# Autodesk Inventor assembly: !drive_pod
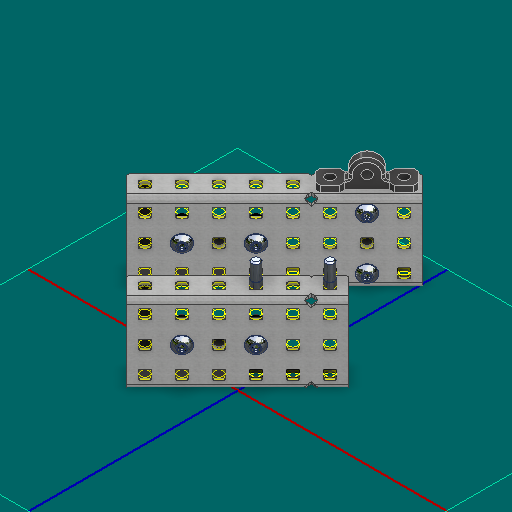
[picture p0: Inventor's stored thumbnail of the model, 512x512]
Saved by Autodesk Inventor 2025 (Build 290162000, 162)
## iProperties
Created: 2024-08-16
Part Number: !drive_pod
Document SubType Name: Assembly
Designer: averey
Author: averey
## Documents named in this file (12)
- C:\Users\avere\vex_robotics_high_stakes\hardware\cad\ATLAS\chassis\drive_pod\structure.iam
- C:\Users\avere\vex_robotics_high_stakes\hardware\cad\VEX-CAD-Inventor\Structure\C Channel\Aluminum 1x3x1\Alu C 1x3x1x6.ipt
- C:\Users\avere\vex_robotics_high_stakes\hardware\cad\_quick_assemblies\bearing_flat_w_hardware.iam
- C:\Users\avere\vex_robotics_high_stakes\hardware\cad\VEX-CAD-Inventor\Structure\C Channel\Aluminum 1x3x1\Alu C 1x3x1x8.ipt
- C:\Users\avere\vex_robotics_high_stakes\hardware\cad\VEX-CAD-Inventor\Motion\Spacers\Spacer Nylon .375 OD.ipt
- C:\Users\avere\vex_robotics_high_stakes\hardware\cad\VEX-CAD-Inventor\Motion\Spacers\Spacer Nylon .375 OD\NSpacer .375 OD x .500.ipt
- C:\Users\avere\vex_robotics_high_stakes\hardware\cad\VEX-CAD-Inventor\Motion\Spacers\Spacer Nylon .375 OD\NSpacer .375 OD x .125.ipt
- C:\Users\avere\vex_robotics_high_stakes\hardware\cad\VEX-CAD-Inventor\Motion\Shaft LS\Bearing Flat Low Profile.ipt
- C:\Users\avere\vex_robotics_high_stakes\hardware\cad\VEX-CAD-Inventor\Structure\Hardware\Nut Thin Nylock.ipt
- C:\Users\avere\vex_robotics_high_stakes\hardware\cad\VEX-CAD-Inventor\Motion\Shaft LS\LS Pillow Bearing Block.ipt
- C:\Users\avere\vex_robotics_high_stakes\hardware\cad\VEX-CAD-Inventor\Structure\Hardware\Screw Shoulder Robosource\SScrew Shoulder Smooth .500 x .18.ipt
- C:\Users\avere\vex_robotics_high_stakes\hardware\cad\VEX-CAD-Inventor\Structure\Hardware\Screw Shoulder Robosource.ipt
## Components (18 placed, 9 different names)
1. Alu C 1x3x1x6:1 — Mate:1, Mate:2, Angle:1, Angle:2, Insert:1, Mate:3, Insert:2, Mate:4, Insert:27, Insert:34, Insert:35
2. bearing_flat_w_hardware:1 [sub-assembly] — Insert:1, Mate:3
3. Alu C 1x3x1x8:1 — Insert:2, Mate:4, Insert:18, Insert:20, Mate:11, Insert:30, Mate:12, Insert:32, Mate:14, Insert:33, Mate:15
4. NSpacer .375 OD x .500:5 — Insert:18
5. NSpacer .375 OD x .500:6 — Insert:19
6. NSpacer .375 OD x .125:7 — Insert:19, Insert:23
7. Bearing Flat Low Profile:1 — Insert:20, Mate:11, Insert:23, Insert:28
8. NSpacer .375 OD x .500:8 — Insert:27
9. NSpacer .375 OD x .500:9
10. NSpacer .375 OD x .125:10
11. Bearing Flat Low Profile:2 — Insert:29
12. Nut Thin Nylock:1 — Insert:28
13. Nut Thin Nylock:2 — Insert:29
14. bearing_flat_w_hardware:2 [sub-assembly] — Insert:30, Mate:12
15. LS Pillow Bearing Block:2 — Insert:32, Mate:14
16. bearing_flat_w_hardware:3 [sub-assembly] — Insert:33, Mate:15
17. SScrew Shoulder Smooth .500 x .18:1 — Insert:34
18. SScrew Shoulder Smooth .500 x .18:2 — Insert:35
## Relationships (28: Insert 18, Mate 8, Angle 2)
- Mate:1: Alu C 1x3x1x6:1
- Mate:2 (-6.35 mm): Alu C 1x3x1x6:1
- Angle:1 (0 deg): Alu C 1x3x1x6:1
- Angle:2 (45 deg): Alu C 1x3x1x6:1
- Insert:1: Alu C 1x3x1x6:1 ↔ bearing_flat_w_hardware:1
- Mate:3: Alu C 1x3x1x6:1 ↔ bearing_flat_w_hardware:1
- Insert:2 (58.7375 mm): Alu C 1x3x1x6:1 ↔ Alu C 1x3x1x8:1
- Mate:4: Alu C 1x3x1x6:1 ↔ Alu C 1x3x1x8:1
- [Insert]: NSpacer .375 OD x .500:5 ↔ NSpacer .375 OD x .500:6
- Insert:18: Alu C 1x3x1x8:1 ↔ NSpacer .375 OD x .500:5
- Insert:19: NSpacer .375 OD x .500:6 ↔ NSpacer .375 OD x .125:7
- Insert:20: Alu C 1x3x1x8:1 ↔ Bearing Flat Low Profile:1
- Mate:11: Alu C 1x3x1x8:1 ↔ Bearing Flat Low Profile:1
- Insert:23 (1.27 mm): NSpacer .375 OD x .125:7 ↔ Bearing Flat Low Profile:1
- [Insert]: NSpacer .375 OD x .500:8 ↔ NSpacer .375 OD x .500:9
- [Insert]: NSpacer .375 OD x .500:9 ↔ NSpacer .375 OD x .125:10
- [Insert] (1.27 mm): NSpacer .375 OD x .125:10 ↔ Bearing Flat Low Profile:2
- Insert:27: Alu C 1x3x1x6:1 ↔ NSpacer .375 OD x .500:8
- Insert:28 (1.27 mm): Bearing Flat Low Profile:1 ↔ Nut Thin Nylock:1
- Insert:29 (1.27 mm): Bearing Flat Low Profile:2 ↔ Nut Thin Nylock:2
- Insert:30: Alu C 1x3x1x8:1 ↔ bearing_flat_w_hardware:2
- Mate:12: Alu C 1x3x1x8:1 ↔ bearing_flat_w_hardware:2
- Insert:32: Alu C 1x3x1x8:1 ↔ LS Pillow Bearing Block:2
- Mate:14: Alu C 1x3x1x8:1 ↔ LS Pillow Bearing Block:2
- Insert:33: Alu C 1x3x1x8:1 ↔ bearing_flat_w_hardware:3
- Mate:15: Alu C 1x3x1x8:1 ↔ bearing_flat_w_hardware:3
- Insert:34: Alu C 1x3x1x6:1 ↔ SScrew Shoulder Smooth .500 x .18:1
- Insert:35: Alu C 1x3x1x6:1 ↔ SScrew Shoulder Smooth .500 x .18:2
## Named parameters: d39_d36 = 0 mm, d57_d39_d36 = 0 mm, d58_d51 = 0 mm, d59_d56 = 1.27 mm
